# Autodesk Inventor assembly: CO-0-1-BatteryUnit
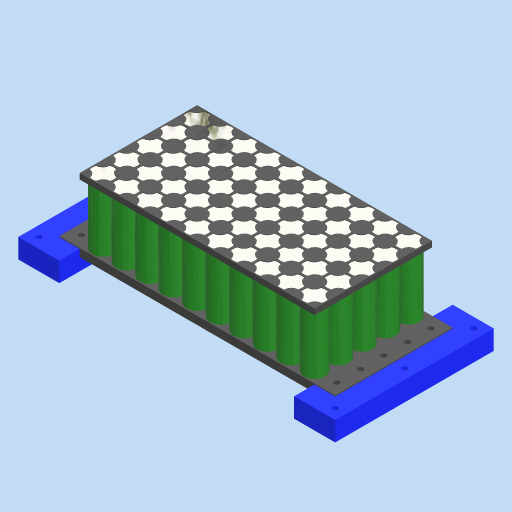
[picture p0: Inventor's stored thumbnail of the model, 512x512]
Saved by Autodesk Inventor 2023 (Build 270158000, 158)
## iProperties
Created: 2023-01-22
Part Number: CO-0-1-BatteryUnit
Document SubType Name: Assembly
Designer: asach
Author: asach
## Documents named in this file (5)
- C:\Github\BehrendURC\CAD\Controls\CO-0-1-BatteryUnit.iam
- C:\Github\BehrendURC\CAD\Controls\CO-2-1_CellSpacerBottom.ipt
- C:\Github\BehrendURC\CAD\Controls\CO-1-1-BatteryCell.ipt
- C:\Github\BehrendURC\CAD\Controls\CO-1-1_CellSpacer10by5.ipt
- C:\Github\BehrendURC\CAD\Controls\CO-1-1-CellSpacerMount.ipt
## Components (54 placed, 4 different names)
1. CO-2-1_CellSpacerBottom:1 — Mate:1, Mate:2, Mate:6, Mate:7, Mate:8, Mate:9, Mate:10, Mate:11
2. CO-1-1_CellSpacer10by5:1 — Mate:3, Mate:4, Mate:5
3. CO-1-1-CellSpacerMount:1 — Mate:6, Mate:7, Mate:8
4. CO-1-1-CellSpacerMount:2 — Mate:9, Mate:10, Mate:11
5. CO-1-1-BatteryCell:1 — Mate:1, Mate:2, Mate:5
6. CO-1-1-BatteryCell:2
7. CO-1-1-BatteryCell:3
8. CO-1-1-BatteryCell:4
9. CO-1-1-BatteryCell:5
10. CO-1-1-BatteryCell:6
11. CO-1-1-BatteryCell:7
12. CO-1-1-BatteryCell:8
13. CO-1-1-BatteryCell:9
14. CO-1-1-BatteryCell:10
15. CO-1-1-BatteryCell:11
16. CO-1-1-BatteryCell:12
17. CO-1-1-BatteryCell:13
18. CO-1-1-BatteryCell:14
19. CO-1-1-BatteryCell:15
20. CO-1-1-BatteryCell:16
21. CO-1-1-BatteryCell:17
22. CO-1-1-BatteryCell:18
23. CO-1-1-BatteryCell:19
24. CO-1-1-BatteryCell:20
25. CO-1-1-BatteryCell:21
26. CO-1-1-BatteryCell:22
27. CO-1-1-BatteryCell:23
28. CO-1-1-BatteryCell:24
29. CO-1-1-BatteryCell:25
30. CO-1-1-BatteryCell:26
31. CO-1-1-BatteryCell:27
32. CO-1-1-BatteryCell:28
33. CO-1-1-BatteryCell:29
34. CO-1-1-BatteryCell:30
35. CO-1-1-BatteryCell:31
36. CO-1-1-BatteryCell:32
37. CO-1-1-BatteryCell:33
38. CO-1-1-BatteryCell:34
39. CO-1-1-BatteryCell:35
40. CO-1-1-BatteryCell:36
41. CO-1-1-BatteryCell:37
42. CO-1-1-BatteryCell:38
43. CO-1-1-BatteryCell:39
44. CO-1-1-BatteryCell:40
45. CO-1-1-BatteryCell:41
46. CO-1-1-BatteryCell:42
47. CO-1-1-BatteryCell:43
48. CO-1-1-BatteryCell:44
49. CO-1-1-BatteryCell:45
50. CO-1-1-BatteryCell:46
51. CO-1-1-BatteryCell:47
52. CO-1-1-BatteryCell:48
53. CO-1-1-BatteryCell:49
54. CO-1-1-BatteryCell:50 — Mate:3, Mate:4
## Component patterns: (50 elements, first: CO-1-1-BatteryCell:1)
## Relationships (11: Mate 11)
- Mate:1: CO-2-1_CellSpacerBottom:1 ↔ CO-1-1-BatteryCell:1
- Mate:2: CO-2-1_CellSpacerBottom:1 ↔ CO-1-1-BatteryCell:1
- Mate:3: CO-1-1_CellSpacer10by5:1 ↔ CO-1-1-BatteryCell:50
- Mate:4: CO-1-1_CellSpacer10by5:1 ↔ CO-1-1-BatteryCell:50
- Mate:5: CO-1-1_CellSpacer10by5:1 ↔ CO-1-1-BatteryCell:1
- Mate:6: CO-2-1_CellSpacerBottom:1 ↔ CO-1-1-CellSpacerMount:1
- Mate:7: CO-2-1_CellSpacerBottom:1 ↔ CO-1-1-CellSpacerMount:1
- Mate:8: CO-2-1_CellSpacerBottom:1 ↔ CO-1-1-CellSpacerMount:1
- Mate:9: CO-2-1_CellSpacerBottom:1 ↔ CO-1-1-CellSpacerMount:2
- Mate:10: CO-2-1_CellSpacerBottom:1 ↔ CO-1-1-CellSpacerMount:2
- Mate:11: CO-2-1_CellSpacerBottom:1 ↔ CO-1-1-CellSpacerMount:2
